# Autodesk Inventor assembly: Assembly1
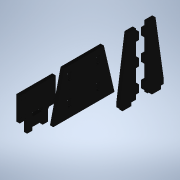
[picture p0: Inventor's stored thumbnail of the model, 180x180]
Saved by Autodesk Inventor 2021 (Build 250183000, 183)
## iProperties
Created: 2020-11-26
Part Number: Assembly1
Document SubType Name: Assembly
Designer: deli
Author: deli
## Documents named in this file (5)
- C:\Users\deli\OneDrive - Eastside Preparatory School\FTC\Ultamite Goal\9884\JSun Chassi\Assembly1.iam
- C:\Users\deli\OneDrive - Eastside Preparatory School\Personal\CNC\Upgrades to Maslow\Z-Axis Carriage Plate.ipt
- C:\Users\deli\OneDrive - Eastside Preparatory School\Personal\CNC\Upgrades to Maslow\Z-Axis Gusset(Mirror).ipt
- C:\Users\deli\OneDrive - Eastside Preparatory School\Personal\CNC\Upgrades to Maslow\Z-Axis Gusset.ipt
- C:\Users\deli\OneDrive - Eastside Preparatory School\Personal\CNC\Upgrades to Maslow\Z-Axis Spine.ipt
## Components (4 placed, 4 different names)
1. Z-Axis Carriage Plate:1 — Flush:3
2. Z-Axis Gusset(Mirror):1 — Flush:1
3. Z-Axis Gusset:1 — Flush:2
4. Z-Axis Spine:1 — Flush:1, Flush:2, Flush:3
## Relationships (3: Flush 3)
- Flush:1: Z-Axis Gusset(Mirror):1 ↔ Z-Axis Spine:1
- Flush:2: Z-Axis Gusset:1 ↔ Z-Axis Spine:1
- Flush:3: Z-Axis Carriage Plate:1 ↔ Z-Axis Spine:1
